# Autodesk Inventor assembly: 739282
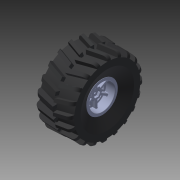
[picture p0: Inventor's stored thumbnail of the model, 180x180]
Saved by Autodesk Inventor 2016 SP1 (Build 200210100, 210)
## iProperties
Category: Add-on Components
Company: Autodesk Inc.
Created: 2014-11-26
Part Number: 739282
Document SubType Name: Assembly
Designer: Tetrix
Catalog Web Link: http://www.tetrixrobotics.com/Wheels/TETRIX_All-Terrain_Tire
Vendor: Tetrix
Author: Autodesk Inc.
## Documents named in this file (3)
- D:\FIRST\FTC\FTC KOP 2016\Tetrix\Tetrix_739282.iam
- D:\FIRST\FTC\FTC KOP 2016\Tetrix\Tetrix_739282_Hub.ipt
- D:\FIRST\FTC\FTC KOP 2016\Tetrix\Tetrix_739282_Tire.ipt
## Components (2 placed, 2 different names)
1. Tetrix_739282_Hub:1 — Insert:1
2. Tetrix_739282_Tire:1 — Insert:1
## Relationships (1: Insert 1)
- Insert:1: Tetrix_739282_Hub:1 ↔ Tetrix_739282_Tire:1
